# Autodesk Inventor assembly: LaundryRobot_v01
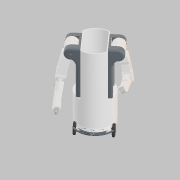
[picture p0: Inventor's stored thumbnail of the model, 180x180]
Saved by Autodesk Inventor 2017 (Build 210142000, 142)
## iProperties
Created: 2017-03-11
Part Number: LaundryRobot_v01
Document SubType Name: Assembly
Designer: zallen
Author: zallen
## Documents named in this file (3)
- C:\Users\zallen\Documents\GitHub\cr-laundry-robot\LaundryRobot_v01.iam
- C:\Users\zallen\Documents\GitHub\cr-laundry-robot\src\Base\Base.iam
- C:\Users\zallen\Documents\GitHub\cr-laundry-robot\src\Body\Body.iam
## Components (2 placed, 2 different names)
1. Base:1 [sub-assembly] — Mate:1, Mate:2
2. Body:1 [sub-assembly] — Mate:1, Mate:2
## Relationships (2: Mate 2)
- Mate:1: Base:1 ↔ Body:1
- Mate:2: Base:1 ↔ Body:1
